# Autodesk Inventor assembly: Ensamble_Llanta
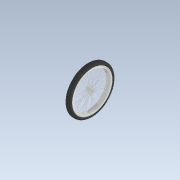
[picture p0: Inventor's stored thumbnail of the model, 180x180]
Saved by Autodesk Inventor 2021 (Build 250183000, 183)
## iProperties
Created: 2021-04-15
Part Number: Ensamble_Llanta
Document SubType Name: Assembly
Designer: j2seb
Author: j2seb
## Documents named in this file (6)
- C:\Git\Proyecto_APM\02 Inventor\Ensamble_Llanta.iam
- C:\Git\Proyecto_APM\02 Inventor\manzana1.ipt
- C:\Git\Proyecto_APM\02 Inventor\protector.ipt
- C:\Git\Proyecto_APM\02 Inventor\cubierta.ipt
- C:\Git\Proyecto_APM\02 Inventor\neumatico.ipt
- C:\Git\Proyecto_APM\02 Inventor\cinta_protectora.ipt
## Components (5 placed, 5 different names)
1. manzana1:1
2. protector:1
3. cubierta:1
4. neumatico:1 — Nivelación:1
5. cinta_protectora:1 — Nivelación:2
## Relationships (2: Flush 2)
- Nivelación:1 [Flush]: neumatico:1
- Nivelación:2 [Flush]: cinta_protectora:1
